# Autodesk Inventor assembly: controller case
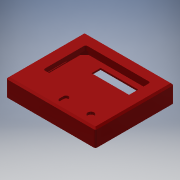
[picture p0: Inventor's stored thumbnail of the model, 180x180]
Saved by Autodesk Inventor 2018 (Build 220112000, 112)
## iProperties
Created: 2017-11-16
Part Number: controller case
Material: Generisch
Document SubType Name: Assembly
Designer: Till
Author: Till
## Documents named in this file (3)
- C:\Users\Till\Dropbox\Ultibox\ultibox\cad\RepRap Full Graphic Smart Controller\controller case.iam
- C:\Users\Till\Dropbox\Ultibox\ultibox\cad\RepRap Full Graphic Smart Controller\case front.ipt
- C:\Users\Till\Dropbox\Ultibox\ultibox\cad\RepRap Full Graphic Smart Controller\case rear.ipt
## Components (2 placed, 2 different names)
1. case front:1 — Fluchtend:1, Fluchtend:2, Passend:1, Passend:2
2. case rear:1 — Passend:2
## Relationships (4: Flush 2, Mate 2)
- Fluchtend:1 [Flush]: case front:1
- Fluchtend:2 [Flush]: case front:1
- Passend:1 [Mate]: case front:1
- Passend:2 [Mate]: case front:1 ↔ case rear:1
